# Autodesk Inventor assembly: Assembly2
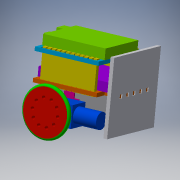
[picture p0: Inventor's stored thumbnail of the model, 180x180]
Saved by Autodesk Inventor 2016 (Build 200138000, 138)
## iProperties
Created: 2017-09-14
Part Number: Assembly2
Document SubType Name: Assembly
Designer: student
Author: student
## Documents named in this file (12)
- D:\sumo bot\Assembly2.iam
- D:\sumo bot\msheehan_motor_mount.ipt
- D:\sumo bot\msheehan_motor.ipt
- D:\sumo bot\msheehan_wheel_small.ipt
- D:\sumo bot\msheehan_battery.ipt
- D:\sumo bot\msheehan_small_breadboard.ipt
- D:\sumo bot\msheehan_ring_small.ipt
- D:\sumo bot\frame\Frame.ipt
- D:\sumo bot\frame\frame_front.ipt
- D:\sumo bot\frame\frame_side.ipt
- D:\sumo bot\frame\frame_top.ipt
- D:\sumo bot\msheehan_uno_board.ipt
## Components (16 placed, 11 different names)
1. msheehan_motor_mount:1 — Rigid:4, Rigid:10
2. msheehan_motor_mount:2 — Rigid:3, Rigid:11
3. msheehan_motor:1 — Rigid:4, Rotational:1
4. msheehan_motor:2 — Rigid:3, Rotational:2
5. msheehan_wheel_small:1 — Rotational:2, Rigid:9
6. msheehan_wheel_small:2 — Rotational:1, Rigid:8
7. msheehan_battery:1 — Rigid:17
8. msheehan_small_breadboard:1 — Rigid:16
9. msheehan_ring_small:1 — Rigid:8
10. msheehan_ring_small:2 — Rigid:9
11. Frame:1 — Rigid:10, Rigid:11, Rigid:12, Rigid:14, Rigid:16, Rigid:17, Rigid:20
12. frame_side:1 — Rigid:14
13. frame_side:2 — Rigid:12, Rigid:18
14. frame_top:1 — Rigid:18, Rigid:19
15. msheehan_uno_board:1 — Rigid:19
16. frame_front:1 — Rigid:20
## Relationships (15: WeldJoint 13, RevoluteJoint 2)
- Rigid:3 [WeldJoint]: msheehan_motor_mount:2 ↔ msheehan_motor:2
- Rigid:4 [WeldJoint]: msheehan_motor_mount:1 ↔ msheehan_motor:1
- Rotational:1 [RevoluteJoint]: msheehan_motor:1 ↔ msheehan_wheel_small:2
- Rotational:2 [RevoluteJoint]: msheehan_motor:2 ↔ msheehan_wheel_small:1
- Rigid:8 [WeldJoint]: msheehan_wheel_small:2 ↔ msheehan_ring_small:1
- Rigid:9 [WeldJoint]: msheehan_wheel_small:1 ↔ msheehan_ring_small:2
- Rigid:10 [WeldJoint]: msheehan_motor_mount:1 ↔ Frame:1
- Rigid:11 [WeldJoint]: msheehan_motor_mount:2 ↔ Frame:1
- Rigid:12 [WeldJoint]: Frame:1 ↔ frame_side:2
- Rigid:14 [WeldJoint]: Frame:1 ↔ frame_side:1
- Rigid:16 [WeldJoint]: msheehan_small_breadboard:1 ↔ Frame:1
- Rigid:17 [WeldJoint]: msheehan_battery:1 ↔ Frame:1
- Rigid:18 [WeldJoint]: frame_side:2 ↔ frame_top:1
- Rigid:19 [WeldJoint]: frame_top:1 ↔ msheehan_uno_board:1
- Rigid:20 [WeldJoint]: Frame:1 ↔ frame_front:1
